# Autodesk Inventor assembly: BEARING SYSTEM
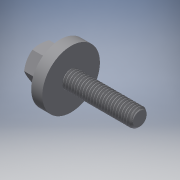
[picture p0: Inventor's stored thumbnail of the model, 180x180]
Saved by Autodesk Inventor 2018 (Build 220112000, 112)
## iProperties
Created: 2018-10-15
Part Number: BEARING SYSTEM
Material: Genérico
Document SubType Name: Assembly
Designer: Toshiba
Author: Toshiba
## Documents named in this file (4)
- C:\U\Semestre Primavera 2018\Diseño de sistemas mecánicos\CNC\DiseñoCNC\Gantry\BEARING SYSTEM.iam
- C:\U\Semestre Primavera 2018\Diseño de sistemas mecánicos\CNC\DiseñoCNC\Gantry\HEX SCREW M8.ipt
- C:\U\Semestre Primavera 2018\Diseño de sistemas mecánicos\CNC\DiseñoCNC\Gantry\THIN HEX NUT M8.ipt
- C:\U\Semestre Primavera 2018\Diseño de sistemas mecánicos\CNC\DiseñoCNC\Gantry\BEARING WHEEL.ipt
## Components (3 placed, 3 different names)
1. HEX SCREW M8:1 — Insertar:1, Ángulo:1
2. THIN HEX NUT M8:1 — Insertar:1, Ángulo:1, Insertar:2
3. BEARING WHEEL:1 — Insertar:2
## Relationships (3: Insert 2, Angle 1)
- Insertar:1: HEX SCREW M8:1 ↔ THIN HEX NUT M8:1
- Ángulo:1 [Angle] (0 deg): HEX SCREW M8:1 ↔ THIN HEX NUT M8:1
- Insertar:2: THIN HEX NUT M8:1 ↔ BEARING WHEEL:1
